# Autodesk Inventor assembly: 리프트_회전부_WORK
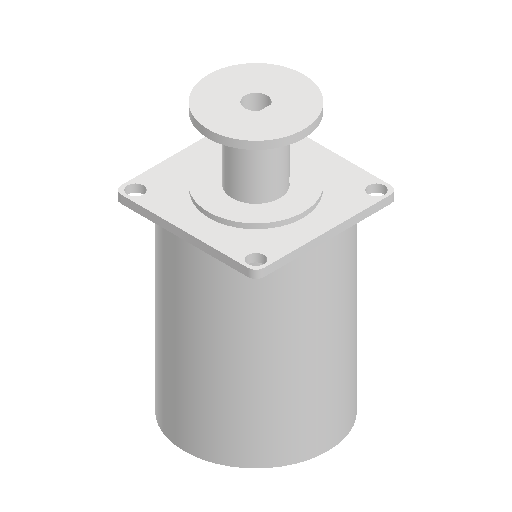
[picture p0: Inventor's stored thumbnail of the model, 512x512]
Saved by Autodesk Inventor 2027 (Build 310192000, 192)
## iProperties
Created: 2026-09-20
Part Number: 리프트_회전부_WORK
Document SubType Name: Assembly
Designer: Kwon
Author: Kwon
## Documents named in this file (5)
- C:\Users\User\Desktop\4_권도영\졸업작품\INVENTOR\리프트_회전부\리프트_회전부_WORK.iam
- C:\Users\User\Desktop\4_권도영\졸업작품\INVENTOR\리프트_회전부\모터.ipt
- C:\Users\User\Desktop\4_권도영\졸업작품\INVENTOR\리프트_회전부\도르래.ipt
- C:\Users\User\Desktop\4_권도영\졸업작품\INVENTOR\리프트_회전부\안쪽_베어링 고정부.ipt
- C:\Users\User\Desktop\4_권도영\졸업작품\INVENTOR\리프트_회전부\베어링.ipt
## Components (4 placed, 4 different names)
1. 모터:1 — 삽입:1, 삽입:5, 삽입:6, 삽입:7, 삽입:8, 삽입:9
2. 도르래:1 — 삽입:1, 삽입:2, 삽입:5, 삽입:6, 삽입:7, 삽입:8, 삽입:9
3. 안쪽_베어링 고정부:1 — 삽입:2, 삽입:3, 삽입:4, 메이트:1
4. 베어링:1 — 삽입:3, 삽입:4, 메이트:1
## Relationships (10: Insert 9, Mate 1)
- 삽입:1 [Insert] (40 mm): 모터:1 ↔ 도르래:1
- 삽입:2 [Insert] (40 mm): 도르래:1 ↔ 안쪽_베어링 고정부:1
- 삽입:3 [Insert] (40 mm): 안쪽_베어링 고정부:1 ↔ 베어링:1
- 삽입:4 [Insert]: 안쪽_베어링 고정부:1 ↔ 베어링:1
- 메이트:1 [Mate]: 안쪽_베어링 고정부:1 ↔ 베어링:1
- 삽입:5 [Insert]: 모터:1 ↔ 도르래:1
- 삽입:6 [Insert]: 모터:1 ↔ 도르래:1
- 삽입:7 [Insert]: 모터:1 ↔ 도르래:1
- 삽입:8 [Insert]: 모터:1 ↔ 도르래:1
- 삽입:9 [Insert]: 모터:1 ↔ 도르래:1
